# Autodesk Inventor assembly: 足回り
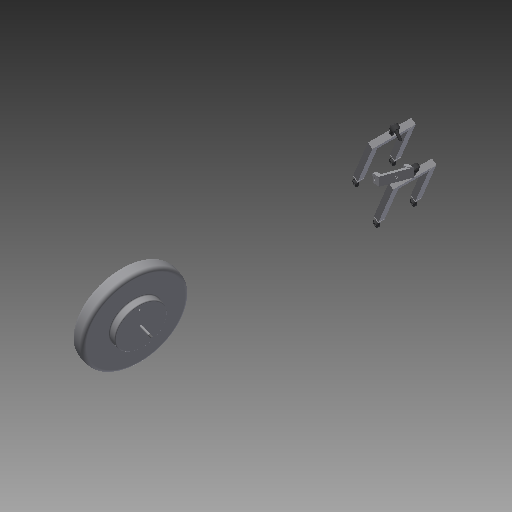
[picture p0: Inventor's stored thumbnail of the model, 512x512]
Saved by Autodesk Inventor 2018 (Build 220112000, 112)
## iProperties
Created: 2017-09-10
Part Number: 足回り
Material: 一般
Document SubType Name: Assembly
Designer: mura5
Author: mura5
## Documents named in this file (5)
- C:\Users\Kenta\Documents\workspace\rbbr\cart\足回り.iam
- C:\Users\Kenta\Documents\workspace\rbbr\cart\A.iam
- C:\Users\Kenta\Documents\workspace\rbbr\cart\車輪取り付け部.iam
- C:\Users\Kenta\Documents\workspace\rbbr\cart\前輪.ipt
- C:\Users\Kenta\Documents\workspace\rbbr\cart\前輪シャフト.ipt
## Components (5 placed, 4 different names)
1. A:1 [sub-assembly] — 回転:7, フラッシュ:1, 角度:2
2. A:2 [sub-assembly] — フラッシュ:1, 角度:2
3. 車輪取り付け部:1 [sub-assembly] — 角度:1, 回転:7
4. 前輪:1 — 回転:8
5. 前輪シャフト:1 — 回転:8
## Relationships (5: Angle 2, RevoluteJoint 2, Flush 1)
- 角度:1 [Angle] (180 deg): 車輪取り付け部:1
- 回転:7 [RevoluteJoint]: A:1 ↔ 車輪取り付け部:1
- フラッシュ:1 [Flush]: A:1 ↔ A:2
- 回転:8 [RevoluteJoint]: 前輪:1 ↔ 前輪シャフト:1
- 角度:2 [Angle] (0 deg): A:1 ↔ A:2
